# Autodesk Inventor assembly: PneumaticWheel_am-0970-2
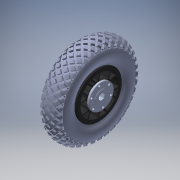
[picture p0: Inventor's stored thumbnail of the model, 180x180]
Saved by Autodesk Inventor 2016 (Build 200138000, 138)
## iProperties
Created: 2011-11-15
Part Number: PneumaticWheel_am-0970-2
Description: STEP AP214
Document SubType Name: Assembly
Designer: gus
Mass: 507.255 g
Surface Area: 2468.36 cm^2
Volume: 469.032 cm^3
Density: 1.08149 g/cm^3
Sending System: SolidWorks 2010
Preprocessor: SwSTEP 2.0
Title: Pneumatic Wheel.STEP
Author: Mark
Revision Number: ANY
## Documents named in this file (4)
- \\Mac\Home\Desktop\2016 robot cad\roller wheels\pnumatic wheel\PneumaticWheel_am-0970-2.iam
- \\Mac\Home\Desktop\2016 robot cad\roller wheels\pnumatic wheel\Tire.ipt
- \\Mac\Home\Desktop\2016 robot cad\roller wheels\pnumatic wheel\Pneumatic Hub.iam
- \\Mac\Home\Desktop\2016 robot cad\roller wheels\am-0096a+500+Hex+Hub+r2.ipt
## Components (3 placed, 3 different names)
1. Tire_1 — Rotational:1
2. Pneumatic Hub_3 [sub-assembly] — Rotational:1, Cylindrical:1, Mate:1, Mate:2
3. am-0096a+500+Hex+Hub+r2:1 — Cylindrical:1, Mate:1, Mate:2
## Relationships (4: Mate 2, RevoluteJoint 1, CylindricalJoint 1)
- Rotational:1 [RevoluteJoint]: Tire_1 ↔ Pneumatic Hub_3
- Cylindrical:1: Pneumatic Hub_3 ↔ am-0096a+500+Hex+Hub+r2:1
- Mate:1: Pneumatic Hub_3 ↔ am-0096a+500+Hex+Hub+r2:1
- Mate:2: Pneumatic Hub_3 ↔ am-0096a+500+Hex+Hub+r2:1
